# Autodesk Inventor assembly: leg_test
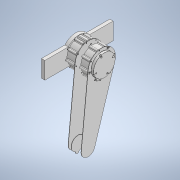
[picture p0: Inventor's stored thumbnail of the model, 180x180]
Saved by Autodesk Inventor 2022.5 (Build 265521000, 521)
## iProperties
Created: 2024-06-26
Part Number: leg_test
Document SubType Name: Assembly
Designer: gakut
Author: gakut
## Documents named in this file (5)
- C:\Users\gakut\Documents\Inventor\leg_test_cad\leg_test.iam
- C:\Users\gakut\Documents\Inventor\leg_test_cad\motor\CyberGear.ipt
- C:\Users\gakut\Documents\Inventor\leg_test_cad\parts\main_plate.ipt
- C:\Users\gakut\Documents\Inventor\leg_test_cad\parts\knee_drive_plate.ipt
- C:\Users\gakut\Documents\Inventor\leg_test_cad\parts\leg_base_plate.ipt
## Components (7 placed, 4 different names)
1. CyberGear:2 — 挿入:2, 挿入:5
2. main_plate:1 — メイト:4, メイト:6, 挿入:5, メイト:7
3. knee_drive_plate:1 — 挿入:2, フラッシュ:1
4. knee_drive_plate:2 — メイト:4, フラッシュ:1
5. leg_base_plate:1 — フラッシュ:2, メイト:5, 挿入:3, メイト:8
6. CyberGear:3 — 挿入:3, 挿入:4
7. main_plate:2 — 挿入:4, メイト:6, メイト:7
## Relationships (11: Mate 5, Insert 4, Flush 2)
- 挿入:2 [Insert]: CyberGear:2 ↔ knee_drive_plate:1
- メイト:4 [Mate]: main_plate:1 ↔ knee_drive_plate:2
- フラッシュ:1 [Flush]: knee_drive_plate:1 ↔ knee_drive_plate:2
- フラッシュ:2 [Flush]: leg_base_plate:1
- メイト:5 [Mate]: leg_base_plate:1
- 挿入:3 [Insert]: leg_base_plate:1 ↔ CyberGear:3
- 挿入:4 [Insert]: CyberGear:3 ↔ main_plate:2
- メイト:6 [Mate]: main_plate:1 ↔ main_plate:2
- 挿入:5 [Insert]: CyberGear:2 ↔ main_plate:1
- メイト:7 [Mate]: main_plate:1 ↔ main_plate:2
- メイト:8 [Mate]: leg_base_plate:1
